# Autodesk Inventor assembly: Stempel
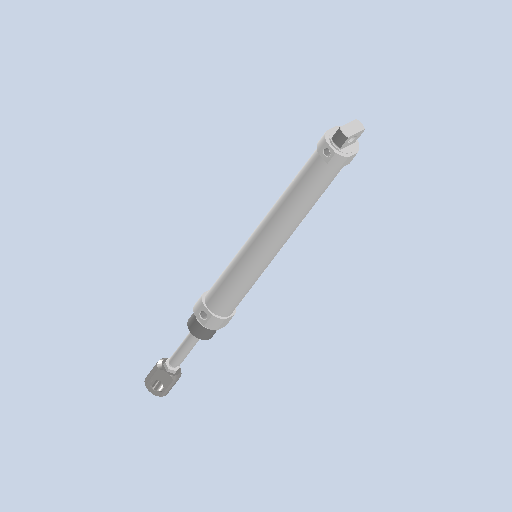
[picture p0: Inventor's stored thumbnail of the model, 512x512]
Saved by Autodesk Inventor 2022 (Build 260153000, 153)
## iProperties
Created: 2022-05-04
Part Number: Stempel
Document SubType Name: Assembly
Designer: patri
Author: patri
## Documents named in this file (5)
- H:\OneDrive - Syddansk Universitet\2. Semester Master\Mekaniske Elementer\Mini Project\2020-10-23\Workspaces\Workspace\Stempel\Stempel.iam
- H:\OneDrive - Syddansk Universitet\2. Semester Master\Mekaniske Elementer\Mini Project\2020-10-23\Workspaces\Workspace\Stempel\193993 DSNU-40-300-P---(A---00--0-KS).ipt
- H:\OneDrive - Syddansk Universitet\2. Semester Master\Mekaniske Elementer\Mini Project\2020-10-23\Workspaces\Workspace\Stempel\193993 DSNU-40-300-P---(A----0-ZR).ipt
- H:\OneDrive - Syddansk Universitet\2. Semester Master\Mekaniske Elementer\Mini Project\2020-10-23\Workspaces\Workspace\Stempel\DIN-439-B - M12x1_25(F).ipt
- H:\OneDrive - Syddansk Universitet\2. Semester Master\Mekaniske Elementer\Mini Project\2020-10-23\Workspaces\Workspace\Stempel\IMS-01-001.ipt
## Components (4 placed, 4 different names)
1. 193993 DSNU-40-300-P---(A---00--0-KS):1 — Cylindrical:1, Flush:2, Mate:2, Mate:4
2. 193993 DSNU-40-300-P---(A----0-ZR):1 — Cylindrical:1
3. DIN-439-B - M12x1_25(F):1 — Flush:2, Mate:3, Mate:4
4. IMS-01-001:1 — Mate:2, Mate:3
## Relationships (5: Mate 3, CylindricalJoint 1, Flush 1)
- Cylindrical:1: 193993 DSNU-40-300-P---(A---00--0-KS):1 ↔ 193993 DSNU-40-300-P---(A----0-ZR):1
- Flush:2 (-10 mm): 193993 DSNU-40-300-P---(A---00--0-KS):1 ↔ DIN-439-B - M12x1_25(F):1
- Mate:2: 193993 DSNU-40-300-P---(A---00--0-KS):1 ↔ IMS-01-001:1
- Mate:3: DIN-439-B - M12x1_25(F):1 ↔ IMS-01-001:1
- Mate:4: 193993 DSNU-40-300-P---(A---00--0-KS):1 ↔ DIN-439-B - M12x1_25(F):1
